# Autodesk Inventor assembly: 000.100 - Манипулятор
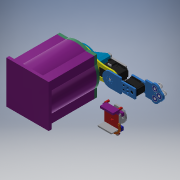
[picture p0: Inventor's stored thumbnail of the model, 180x180]
Saved by Autodesk Inventor 2019 (Build 230136000, 136)
## iProperties
Created: 2020-03-17
Part Number: 000.100 - Манипулятор
Material: Типовые
Document SubType Name: Assembly
Designer: Петров Иван
Author: Петров Иван
## Documents named in this file (7)
- E:\IVAN\Ivan_desktop\Kvantorium\Competitions\INOP_2020\hardware\SCARA(Dynamixels)\000.100 - Манипулятор.iam
- E:\IVAN\Ivan_desktop\Kvantorium\Competitions\INOP_2020\hardware\SCARA(Dynamixels)\000.200 - Основание.iam
- E:\IVAN\Ivan_desktop\Kvantorium\Competitions\INOP_2020\hardware\SCARA(Dynamixels)\000.300 - Рычаг 1.iam
- E:\IVAN\Ivan_desktop\Kvantorium\Competitions\INOP_2020\hardware\SCARA(Dynamixels)\000.400 - Рычаг 2.iam
- E:\IVAN\Ivan_desktop\Kvantorium\Competitions\INOP_2020\hardware\SCARA(Dynamixels)\000.400 - Рычаг 2\000.500 - Подъемная платформа.iam
- E:\IVAN\Ivan_desktop\Kvantorium\Competitions\INOP_2020\hardware\SCARA(Dynamixels)\components\SG90 - Micro Servo 9g - Tower Pro.4.ipt
- E:\IVAN\Ivan_desktop\Kvantorium\Competitions\INOP_2020\hardware\SCARA(Dynamixels)\000.600 - Захват.iam
## Components (6 placed, 6 different names)
1. 000.200 - Основание:1 [sub-assembly] — Совмещение:1, Совмещение:2, Совмещение:3, Угол:1
2. 000.300 - Рычаг 1:1 [sub-assembly] — Совмещение:1, Совмещение:2, Совмещение:3, Совмещение:4, Совмещение:5, Совмещение:6, Угол:1, Угол:2
3. 000.400 - Рычаг 2:1 [sub-assembly] — Совмещение:4, Совмещение:5, Совмещение:6, Угол:2, Совмещение:8, Совмещение:9, Совмещение:15
4. 000.500 - Подъемная платформа:1 [sub-assembly] — Совмещение:8, Совмещение:9, Совмещение:10, Совмещение:11, Совмещение:15
5. SG90 - Micro Servo 9g - Tower Pro.4:1 — Совмещение:10, Совмещение:11, Совмещение:12, Совмещение:13, Совмещение:14
6. 000.600 - Захват:1 [sub-assembly] — Совмещение:12, Совмещение:13, Совмещение:14
## Relationships (16: Mate 14, Angle 2)
- Совмещение:1 [Mate]: 000.200 - Основание:1 ↔ 000.300 - Рычаг 1:1
- Совмещение:2 [Mate]: 000.200 - Основание:1 ↔ 000.300 - Рычаг 1:1
- Совмещение:3 [Mate]: 000.200 - Основание:1 ↔ 000.300 - Рычаг 1:1
- Совмещение:4 [Mate]: 000.300 - Рычаг 1:1 ↔ 000.400 - Рычаг 2:1
- Совмещение:5 [Mate]: 000.300 - Рычаг 1:1 ↔ 000.400 - Рычаг 2:1
- Совмещение:6 [Mate]: 000.300 - Рычаг 1:1 ↔ 000.400 - Рычаг 2:1
- Угол:1 [Angle] (90 deg): 000.200 - Основание:1 ↔ 000.300 - Рычаг 1:1
- Угол:2 [Angle] (0 deg): 000.300 - Рычаг 1:1 ↔ 000.400 - Рычаг 2:1
- Совмещение:8 [Mate]: 000.400 - Рычаг 2:1 ↔ 000.500 - Подъемная платформа:1
- Совмещение:9 [Mate]: 000.400 - Рычаг 2:1 ↔ 000.500 - Подъемная платформа:1
- Совмещение:10 [Mate]: 000.500 - Подъемная платформа:1 ↔ SG90 - Micro Servo 9g - Tower Pro.4:1
- Совмещение:11 [Mate]: 000.500 - Подъемная платформа:1 ↔ SG90 - Micro Servo 9g - Tower Pro.4:1
- Совмещение:12 [Mate]: SG90 - Micro Servo 9g - Tower Pro.4:1 ↔ 000.600 - Захват:1
- Совмещение:13 [Mate]: SG90 - Micro Servo 9g - Tower Pro.4:1 ↔ 000.600 - Захват:1
- Совмещение:14 [Mate]: SG90 - Micro Servo 9g - Tower Pro.4:1 ↔ 000.600 - Захват:1
- Совмещение:15 [Mate]: 000.400 - Рычаг 2:1 ↔ 000.500 - Подъемная платформа:1
